# Autodesk Inventor assembly: body
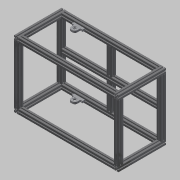
[picture p0: Inventor's stored thumbnail of the model, 180x180]
Saved by Autodesk Inventor 2021.2 (Build 252289000, 289)
## iProperties
Created: 2021-07-09
Part Number: body
Material: 一般
Document SubType Name: Assembly
Designer: gisen
Mass: 47360.5 g
Surface Area: 66475.9 cm^2
Volume: 35407.1 cm^3
Density: 1.3376 g/cm^3
Author: gisen
## Documents named in this file (6)
- C:\Users\gisen\workspace\beetle_inventor_model\body\body.iam
- C:\Users\gisen\workspace\beetle_inventor_model\body\AFS-3030-600.ipt
- C:\Users\gisen\workspace\beetle_inventor_model\body\AFS-3030-360.ipt
- C:\Users\gisen\workspace\beetle_inventor_model\body\AFS-3030-300.ipt
- C:\Users\gisen\workspace\beetle_inventor_model\body\AFS-3030-165.ipt
- C:\Users\gisen\workspace\beetle_inventor_model\body\C-BGHKA6902ZZ-30\C-BGHKA6902ZZ-30.iam
## Components (17 placed, 5 different names)
1. AFS-3030-600:1 — フラッシュ:1, メイト:1, メイト:2, メイト:3, フラッシュ:2, メイト:10, フラッシュ:5, 対称度:1, メイト:14, メイト:20, フラッシュ:10, メイト:33, メイト:34
2. AFS-3030-360:1 — フラッシュ:1, メイト:1, メイト:2, メイト:4, メイト:9, 角度:2, 対称度:2, メイト:12, メイト:15, フラッシュ:8
3. AFS-3030-300:1 — メイト:3, メイト:4, フラッシュ:2
4. AFS-3030-600:2 — メイト:9, 角度:1, 対称度:1, メイト:11, フラッシュ:7, メイト:18, メイト:29, メイト:30
5. AFS-3030-360:2 — メイト:10, フラッシュ:5, 対称度:2, メイト:13
6. AFS-3030-300:2 — メイト:31
7. AFS-3030-300:3 — フラッシュ:6, メイト:13, メイト:14
8. AFS-3030-300:4 — フラッシュ:6, メイト:11, フラッシュ:7, メイト:12, メイト:27, メイト:28, フラッシュ:14
9. AFS-3030-600:3 — メイト:15, フラッシュ:8, メイト:16, フラッシュ:9
10. AFS-3030-165:1 — メイト:17, メイト:18, フラッシュ:9
11. AFS-3030-165:2 — メイト:19, メイト:20, フラッシュ:10
12. AFS-3030-600:4
13. AFS-3030-360:3 — メイト:27
14. AFS-3030-600:5 — メイト:28, フラッシュ:14
15. AFS-3030-360:4
16. C-BGHKA6902ZZ-30:1 [sub-assembly] — メイト:29, メイト:30, メイト:31, メイト:32
17. C-BGHKA6902ZZ-30:2 [sub-assembly] — メイト:32, メイト:33, メイト:34
## Relationships (52: Mate 34, Flush 14, Angle 2, Symmetry 2)
- フラッシュ:1 [Flush]: AFS-3030-600:1 ↔ AFS-3030-360:1
- メイト:1 [Mate]: AFS-3030-600:1 ↔ AFS-3030-360:1
- メイト:2 [Mate]: AFS-3030-600:1 ↔ AFS-3030-360:1
- メイト:3 [Mate]: AFS-3030-600:1 ↔ AFS-3030-300:1
- メイト:4 [Mate]: AFS-3030-360:1 ↔ AFS-3030-300:1
- フラッシュ:2 [Flush]: AFS-3030-600:1 ↔ AFS-3030-300:1
- [Flush]: AFS-3030-600:2 ↔ AFS-3030-360:2
- [Mate]: AFS-3030-600:2 ↔ AFS-3030-360:2
- [Mate]: AFS-3030-600:2 ↔ AFS-3030-360:2
- [Mate]: AFS-3030-600:2 ↔ AFS-3030-300:2
- [Mate]: AFS-3030-360:2 ↔ AFS-3030-300:2
- [Flush]: AFS-3030-600:2 ↔ AFS-3030-300:2
- メイト:9 [Mate]: AFS-3030-360:1 ↔ AFS-3030-600:2
- メイト:10 [Mate]: AFS-3030-600:1 ↔ AFS-3030-360:2
- フラッシュ:5 [Flush]: AFS-3030-600:1 ↔ AFS-3030-360:2
- 角度:1 [Angle] (0 deg): AFS-3030-600:2
- 角度:2 [Angle] (0 deg): AFS-3030-360:1
- 対称度:1 [Symmetry]: AFS-3030-600:1 ↔ AFS-3030-600:2
- 対称度:2 [Symmetry]: AFS-3030-360:1 ↔ AFS-3030-360:2
- フラッシュ:6 [Flush]: AFS-3030-300:3 ↔ AFS-3030-300:4
- メイト:11 [Mate]: AFS-3030-600:2 ↔ AFS-3030-300:4
- フラッシュ:7 [Flush]: AFS-3030-600:2 ↔ AFS-3030-300:4
- メイト:12 [Mate]: AFS-3030-360:1 ↔ AFS-3030-300:4
- メイト:13 [Mate]: AFS-3030-360:2 ↔ AFS-3030-300:3
- メイト:14 [Mate]: AFS-3030-600:1 ↔ AFS-3030-300:3
- メイト:15 [Mate]: AFS-3030-360:1 ↔ AFS-3030-600:3
- フラッシュ:8 [Flush]: AFS-3030-360:1 ↔ AFS-3030-600:3
- メイト:16 [Mate]: AFS-3030-600:3
- メイト:17 [Mate]: AFS-3030-165:1
- メイト:18 [Mate]: AFS-3030-600:2 ↔ AFS-3030-165:1
- フラッシュ:9 [Flush]: AFS-3030-600:3 ↔ AFS-3030-165:1
- メイト:19 [Mate]: AFS-3030-165:2
- メイト:20 [Mate]: AFS-3030-600:1 ↔ AFS-3030-165:2
- フラッシュ:10 [Flush]: AFS-3030-600:1 ↔ AFS-3030-165:2
- [Flush]: AFS-3030-600:4 ↔ AFS-3030-360:3
- [Mate]: AFS-3030-600:4 ↔ AFS-3030-360:3
- [Mate]: AFS-3030-600:4 ↔ AFS-3030-360:3
- [Flush]: AFS-3030-600:5 ↔ AFS-3030-360:4
- [Mate]: AFS-3030-600:5 ↔ AFS-3030-360:4
- [Mate]: AFS-3030-600:5 ↔ AFS-3030-360:4
- [Mate]: AFS-3030-360:3 ↔ AFS-3030-600:5
- [Mate]: AFS-3030-600:4 ↔ AFS-3030-360:4
- [Flush]: AFS-3030-600:4 ↔ AFS-3030-360:4
- メイト:27 [Mate]: AFS-3030-300:4 ↔ AFS-3030-360:3
- メイト:28 [Mate]: AFS-3030-300:4 ↔ AFS-3030-600:5
- フラッシュ:14 [Flush]: AFS-3030-300:4 ↔ AFS-3030-600:5
- メイト:29 [Mate]: AFS-3030-600:2 ↔ C-BGHKA6902ZZ-30:1
- メイト:30 [Mate] (-15 mm): AFS-3030-600:2 ↔ C-BGHKA6902ZZ-30:1
- メイト:31 [Mate] (80 mm): AFS-3030-300:2 ↔ C-BGHKA6902ZZ-30:1
- メイト:32 [Mate]: C-BGHKA6902ZZ-30:1 ↔ C-BGHKA6902ZZ-30:2
- メイト:33 [Mate]: AFS-3030-600:1 ↔ C-BGHKA6902ZZ-30:2
- メイト:34 [Mate] (-15 mm): AFS-3030-600:1 ↔ C-BGHKA6902ZZ-30:2
## Named parameters: d1489_d1485 = 0 mm, d1490_d1486 = 0 mm, d1491_d1487 = 0 mm, d1492_d1488 = 0 mm, d1493_d1483 = 0 mm, d1494_d1484 = 0 mm, d1515_d1485 = 0 mm, d1516_d1489_d1485 = 0 mm, d1517_d1493_d1483 = 0 mm, d1518_d1494_d1484 = 0 mm, d1519_d1495 = 0 mm, d1520_d1496 = 0 mm, d1521_d1497 = 0 mm, d1522_d1483 = 0 mm, d1523_d1484 = 0 mm
